# Autodesk Inventor assembly: assembly
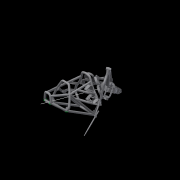
[picture p0: Inventor's stored thumbnail of the model, 180x180]
Saved by Autodesk Inventor 2020 (Build 240168000, 168)
## iProperties
Created: 2020-03-24
Part Number: assembly
Document SubType Name: Assembly
Designer: valer
Author: valer
## Documents named in this file (13)
- C:\Users\valer\Desktop\drummingrobot\src\Robot.iam
- C:\Users\valer\Desktop\drummingrobot\src\Chest.ipt
- C:\Users\valer\Desktop\drummingrobot\src\HeadScaled.ipt
- C:\Users\valer\Desktop\drummingrobot\src\UpperArmServoDynamixelXM430-W350-T.ipt
- C:\Users\valer\Desktop\drummingrobot\src\UpperArm.ipt
- C:\Users\valer\Desktop\drummingrobot\src\UpperArmBracket.ipt
- C:\Users\valer\Desktop\drummingrobot\src\UpperArmMount.ipt
- C:\Users\valer\Desktop\drummingrobot\src\ShoulderChestBracket.ipt
- C:\Users\valer\Desktop\drummingrobot\src\external\ShoulderConnectingRod.ipt
- C:\Users\valer\Desktop\drummingrobot\src\Forearm.ipt
- C:\Users\valer\Desktop\drummingrobot\src\external\Drumstick.ipt
- C:\Users\valer\Desktop\drummingrobot\src\external\ShaftCollar1-2.ipt
- C:\Users\valer\Desktop\drummingrobot\src\external\RodEndFixed.ipt
## Components (25 placed, 12 different names)
1. Chest:1 — Angle:1, Angle:4, Flush:2, Mate:54, Mate:55, Angle:6, Mate:57, Mate:58, Mate:81
2. HeadScaled:1 — Angle:6
3. UpperArmServoDynamixelXM430-W350-T:1 — Angle:1, Mate:10, Mate:11
4. UpperArm:1 — Mate:3, Mate:4, Mate:5, Mate:61, Mate:64
5. UpperArmBracket:1 — Mate:3, Mate:6, Mate:8, Mate:25
6. UpperArmMount:1 — Mate:6, Mate:7, Mate:8, Mate:10, Mate:11, Angle:5, Mate:25, Mate:78
7. UpperArmBracket:2 — Mate:4, Mate:5, Mate:7, Mate:78
8. ShoulderChestBracket:1 — Angle:4, Angle:5, Flush:2, Mate:54, Mate:55, Mate:92, Mate:93, Flush:4, Mate:98, Mate:104, Mate:105, Mate:108, Mate:109
9. ChestConnectingRod:1 — Mate:88, Mate:89
10. ChestConnectingRod:2 — Mate:86, Mate:87
11. ChestConnectingRod:3 — Mate:84, Mate:85
12. ChestConnectingRod:4 — Mate:82, Mate:83
13. ShoulderChestBracket:2 — Mate:57, Mate:58, Mate:81
14. Forearm:1 — Mate:61, Mate:64, Mate:80
15. Drumstick:1 — Mate:79, Flush:3
16. ShaftCollar1/2:1 — Mate:79, Flush:3, Mate:80
17. ShoulderChestBracket:3 — Flush:4, Mate:96, Mate:101, Mate:102, Mate:103, Mate:106, Mate:107
18. RodEnd1/4-1/4-1:1 — Mate:82, Mate:107
19. RodEnd1/4-1/4-1:2 — Mate:83, Mate:92, Mate:109
20. RodEnd1/4-1/4-1:3 — Mate:84, Mate:96, Mate:106
21. RodEnd1/4-1/4-1:4 — Mate:85, Mate:93, Mate:108
22. RodEnd1/4-1/4-1:5 — Mate:86, Mate:102
23. RodEnd1/4-1/4-1:6 — Mate:87, Mate:98, Mate:104
24. RodEnd1/4-1/4-1:7 — Mate:88, Mate:101, Mate:103
25. RodEnd1/4-1/4-1:8 — Mate:89, Mate:105
## Relationships (47: Mate 40, Angle 4, Flush 3)
- Angle:1 (0 deg): Chest:1 ↔ UpperArmServoDynamixelXM430-W350-T:1
- Mate:3: UpperArm:1 ↔ UpperArmBracket:1
- Mate:4: UpperArm:1 ↔ UpperArmBracket:2
- Mate:5: UpperArm:1 ↔ UpperArmBracket:2
- Mate:6: UpperArmBracket:1 ↔ UpperArmMount:1
- Mate:7: UpperArmMount:1 ↔ UpperArmBracket:2
- Mate:8: UpperArmBracket:1 ↔ UpperArmMount:1
- Mate:10: UpperArmServoDynamixelXM430-W350-T:1 ↔ UpperArmMount:1
- Mate:11: UpperArmServoDynamixelXM430-W350-T:1 ↔ UpperArmMount:1
- Angle:4 (0 deg): Chest:1 ↔ ShoulderChestBracket:1
- Angle:5 (0 deg): UpperArmMount:1 ↔ ShoulderChestBracket:1
- Mate:25 (12.7 mm): UpperArmBracket:1 ↔ UpperArmMount:1
- Flush:2: Chest:1 ↔ ShoulderChestBracket:1
- Mate:54 (10.16 mm): Chest:1 ↔ ShoulderChestBracket:1
- Mate:55: Chest:1 ↔ ShoulderChestBracket:1
- Angle:6 (0 deg): Chest:1 ↔ HeadScaled:1
- Mate:57 (10.16 mm): Chest:1 ↔ ShoulderChestBracket:2
- Mate:58: Chest:1 ↔ ShoulderChestBracket:2
- Mate:61: UpperArm:1 ↔ Forearm:1
- Mate:64: UpperArm:1 ↔ Forearm:1
- Mate:78: UpperArmMount:1 ↔ UpperArmBracket:2
- Mate:79: Drumstick:1 ↔ ShaftCollar1/2:1
- Flush:3 (304.8 mm): Drumstick:1 ↔ ShaftCollar1/2:1
- Mate:80: Forearm:1 ↔ ShaftCollar1/2:1
- Mate:81: Chest:1 ↔ ShoulderChestBracket:2
- Mate:82: ChestConnectingRod:4 ↔ RodEnd1/4-1/4-1:1
- Mate:83: ChestConnectingRod:4 ↔ RodEnd1/4-1/4-1:2
- Mate:84: ChestConnectingRod:3 ↔ RodEnd1/4-1/4-1:3
- Mate:85: ChestConnectingRod:3 ↔ RodEnd1/4-1/4-1:4
- Mate:86: ChestConnectingRod:2 ↔ RodEnd1/4-1/4-1:5
- Mate:87: ChestConnectingRod:2 ↔ RodEnd1/4-1/4-1:6
- Mate:88: ChestConnectingRod:1 ↔ RodEnd1/4-1/4-1:7
- Mate:89: ChestConnectingRod:1 ↔ RodEnd1/4-1/4-1:8
- Mate:92: ShoulderChestBracket:1 ↔ RodEnd1/4-1/4-1:2
- Mate:93: ShoulderChestBracket:1 ↔ RodEnd1/4-1/4-1:4
- Flush:4: ShoulderChestBracket:1 ↔ ShoulderChestBracket:3
- Mate:96: ShoulderChestBracket:3 ↔ RodEnd1/4-1/4-1:3
- Mate:98: ShoulderChestBracket:1 ↔ RodEnd1/4-1/4-1:6
- Mate:101: ShoulderChestBracket:3 ↔ RodEnd1/4-1/4-1:7
- Mate:102: ShoulderChestBracket:3 ↔ RodEnd1/4-1/4-1:5
- Mate:103: ShoulderChestBracket:3 ↔ RodEnd1/4-1/4-1:7
- Mate:104: ShoulderChestBracket:1 ↔ RodEnd1/4-1/4-1:6
- Mate:105: ShoulderChestBracket:1 ↔ RodEnd1/4-1/4-1:8
- Mate:106: ShoulderChestBracket:3 ↔ RodEnd1/4-1/4-1:3
- Mate:107: ShoulderChestBracket:3 ↔ RodEnd1/4-1/4-1:1
- Mate:108: ShoulderChestBracket:1 ↔ RodEnd1/4-1/4-1:4
- Mate:109: ShoulderChestBracket:1 ↔ RodEnd1/4-1/4-1:2
